# Autodesk Inventor assembly: Assembly1
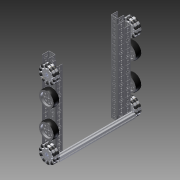
[picture p0: Inventor's stored thumbnail of the model, 180x180]
Saved by Autodesk Inventor 2015 SP1 (Build 190203100, 203)
## iProperties
Created: 2015-03-14
Part Number: Assembly1
Document SubType Name: Assembly
Designer: datenney
Author: datenney
## Documents named in this file (6)
- C:\Users\datenney\Documents\Assembly1.iam
- C:\Users\datenney\Documents\GitHub\CAD\COTSParts\Tetrix\Tetrix Channel 404.25mm.ipt
- C:\Users\datenney\Documents\GitHub\CAD\COTSParts\Tetrix\Tetrix Channel 367.5mm.ipt
- C:\Users\datenney\Documents\GitHub\CAD\COTSParts\Bosch Extrusion\Bosch 20x20 13.75 in.ipt
- C:\Users\datenney\Documents\GitHub\CAD\COTSParts\Tetrix\Tetrix Wheel 3 in omni.ipt
- C:\Users\datenney\Documents\GitHub\CAD\COTSParts\Tetrix\Tetrix wheel 3 in.ipt
## Components (17 placed, 5 different names)
1. Tetrix Channel 404.25mm:1 — Mate:2, Flush:1, Flush:7, Flush:11, Flush:14
2. Tetrix Channel 404.25mm:2 — Mate:1, Flush:7, Flush:11, Flush:12, Flush:13
3. Tetrix Channel 367.5mm_CPY:1 — Mate:1, Mate:16, Mate:17, Mate:18, Mate:19, Mate:24, Mate:25, Mate:28, Mate:29, Flush:10, Flush:12, Flush:13, Flush:16, Mate:34
4. Tetrix Channel 367.5mm_CPY:2 — Mate:2, Flush:1, Mate:14, Mate:15, Mate:20, Mate:21, Mate:22, Mate:23, Mate:26, Mate:27, Flush:14, Flush:15, Flush:17
5. Bosch 20x20 13.75 in:1 — Flush:9, Mate:7, Flush:15, Flush:16, Flush:17, Mate:34
6. Tetrix Wheel 3 in omni:1 — Mate:8, Mate:9, Tangent:2, Mate:29, Mate:30, Rotation:1
7. Tetrix Wheel 3 in omni:2 — Mate:8, Mate:9, Tangent:2, Mate:19
8. Tetrix Wheel 3 in omni:3 — Mate:10, Mate:11, Tangent:3, Mate:15
9. Tetrix Wheel 3 in omni:4 — Mate:10, Mate:11, Tangent:3, Mate:27, Mate:30
10. Tetrix Wheel 3 in omni:5 — Tangent:4, Mate:12, Mate:13, Mate:26, Mate:31
11. Tetrix Wheel 3 in omni:6 — Tangent:4, Mate:12, Mate:13, Mate:14
12. Tetrix Wheel 3 in omni:7 — Mate:5, Mate:6, Tangent:1, Mate:28, Mate:31, Rotation:3
13. Tetrix Wheel 3 in omni:8 — Mate:5, Mate:6, Tangent:1, Mate:16
14. Tetrix wheel 3 in:1 — Mate:18, Mate:24, Mate:33, Rotation:1, Rotation:2
15. Tetrix wheel 3 in:2 — Mate:17, Mate:25, Mate:32, Rotation:2, Rotation:3
16. Tetrix wheel 3 in:3 — Mate:20, Mate:22, Mate:32
17. Tetrix wheel 3 in:4 — Mate:21, Mate:23, Mate:33
## Relationships (50: Mate 32, Flush 11, Tangent 4, RelateRotation 3)
- Mate:1: Tetrix Channel 404.25mm:2 ↔ Tetrix Channel 367.5mm_CPY:1
- Mate:2: Tetrix Channel 404.25mm:1 ↔ Tetrix Channel 367.5mm_CPY:2
- Flush:1 (-21.5519 mm): Tetrix Channel 404.25mm:1 ↔ Tetrix Channel 367.5mm_CPY:2
- Mate:5: Tetrix Wheel 3 in omni:7 ↔ Tetrix Wheel 3 in omni:8
- Mate:6: Tetrix Wheel 3 in omni:7 ↔ Tetrix Wheel 3 in omni:8
- Tangent:1: Tetrix Wheel 3 in omni:7 ↔ Tetrix Wheel 3 in omni:8
- Flush:7: Tetrix Channel 404.25mm:1 ↔ Tetrix Channel 404.25mm:2
- Flush:9: Bosch 20x20 13.75 in:1
- Mate:7: Bosch 20x20 13.75 in:1
- Flush:10: Tetrix Channel 367.5mm_CPY:1
- Mate:8: Tetrix Wheel 3 in omni:1 ↔ Tetrix Wheel 3 in omni:2
- Mate:9: Tetrix Wheel 3 in omni:1 ↔ Tetrix Wheel 3 in omni:2
- Tangent:2: Tetrix Wheel 3 in omni:1 ↔ Tetrix Wheel 3 in omni:2
- Mate:10: Tetrix Wheel 3 in omni:3 ↔ Tetrix Wheel 3 in omni:4
- Mate:11: Tetrix Wheel 3 in omni:3 ↔ Tetrix Wheel 3 in omni:4
- Tangent:3: Tetrix Wheel 3 in omni:3 ↔ Tetrix Wheel 3 in omni:4
- Tangent:4: Tetrix Wheel 3 in omni:5 ↔ Tetrix Wheel 3 in omni:6
- Mate:12: Tetrix Wheel 3 in omni:5 ↔ Tetrix Wheel 3 in omni:6
- Mate:13: Tetrix Wheel 3 in omni:5 ↔ Tetrix Wheel 3 in omni:6
- Mate:14 (2.54 mm): Tetrix Channel 367.5mm_CPY:2 ↔ Tetrix Wheel 3 in omni:6
- Mate:15 (2.54 mm): Tetrix Channel 367.5mm_CPY:2 ↔ Tetrix Wheel 3 in omni:3
- Mate:16 (2.54 mm): Tetrix Channel 367.5mm_CPY:1 ↔ Tetrix Wheel 3 in omni:8
- Mate:17 (2.54 mm): Tetrix Channel 367.5mm_CPY:1 ↔ Tetrix wheel 3 in:2
- Mate:18 (2.54 mm): Tetrix Channel 367.5mm_CPY:1 ↔ Tetrix wheel 3 in:1
- Mate:19 (2.54 mm): Tetrix Channel 367.5mm_CPY:1 ↔ Tetrix Wheel 3 in omni:2
- Mate:20 (2.54 mm): Tetrix Channel 367.5mm_CPY:2 ↔ Tetrix wheel 3 in:3
- Mate:21 (2.54 mm): Tetrix Channel 367.5mm_CPY:2 ↔ Tetrix wheel 3 in:4
- Mate:22: Tetrix Channel 367.5mm_CPY:2 ↔ Tetrix wheel 3 in:3
- Mate:23: Tetrix Channel 367.5mm_CPY:2 ↔ Tetrix wheel 3 in:4
- Mate:24: Tetrix Channel 367.5mm_CPY:1 ↔ Tetrix wheel 3 in:1
- Mate:25: Tetrix Channel 367.5mm_CPY:1 ↔ Tetrix wheel 3 in:2
- Mate:26: Tetrix Channel 367.5mm_CPY:2 ↔ Tetrix Wheel 3 in omni:5
- Mate:27: Tetrix Channel 367.5mm_CPY:2 ↔ Tetrix Wheel 3 in omni:4
- Mate:28: Tetrix Channel 367.5mm_CPY:1 ↔ Tetrix Wheel 3 in omni:7
- Mate:29: Tetrix Channel 367.5mm_CPY:1 ↔ Tetrix Wheel 3 in omni:1
- Mate:30: Tetrix Wheel 3 in omni:1 ↔ Tetrix Wheel 3 in omni:4
- Mate:31: Tetrix Wheel 3 in omni:5 ↔ Tetrix Wheel 3 in omni:7
- Mate:32: Tetrix wheel 3 in:2 ↔ Tetrix wheel 3 in:3
- Mate:33: Tetrix wheel 3 in:1 ↔ Tetrix wheel 3 in:4
- Rotation:1 [RelateRotation] (1 ul): Tetrix Wheel 3 in omni:1 ↔ Tetrix wheel 3 in:1
- Rotation:2 [RelateRotation] (1 ul): Tetrix wheel 3 in:1 ↔ Tetrix wheel 3 in:2
- Rotation:3 [RelateRotation] (1 ul): Tetrix Wheel 3 in omni:7 ↔ Tetrix wheel 3 in:2
- Flush:11: Tetrix Channel 404.25mm:1 ↔ Tetrix Channel 404.25mm:2
- Flush:12 (-21.5519 mm): Tetrix Channel 404.25mm:2 ↔ Tetrix Channel 367.5mm_CPY:1
- Flush:13: Tetrix Channel 404.25mm:2 ↔ Tetrix Channel 367.5mm_CPY:1
- Flush:14: Tetrix Channel 404.25mm:1 ↔ Tetrix Channel 367.5mm_CPY:2
- Flush:15: Tetrix Channel 367.5mm_CPY:2 ↔ Bosch 20x20 13.75 in:1
- Flush:16: Tetrix Channel 367.5mm_CPY:1 ↔ Bosch 20x20 13.75 in:1
- Flush:17: Tetrix Channel 367.5mm_CPY:2 ↔ Bosch 20x20 13.75 in:1
- Mate:34: Tetrix Channel 367.5mm_CPY:1 ↔ Bosch 20x20 13.75 in:1
